# Autodesk Inventor assembly: basic c-channel design
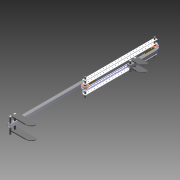
[picture p0: Inventor's stored thumbnail of the model, 180x180]
Saved by Autodesk Inventor 2011 (Build 150239000, 239)
## iProperties
Created: 2013-01-27
Part Number: basic c-channel design
Document SubType Name: Assembly
Designer: Danny
Author: Danny
## Documents named in this file (18)
- C:\Users\Danny\Documents\GitHub\2013CAD\2013 robot\hybrid climber designs\spiderfork\basic c-channel design.iam
- C:\Users\Danny\Documents\GitHub\2013CAD\2013 robot\hybrid climber designs\spiderfork\c-channel (24 in with .5 in holes).ipt
- C:\Users\Danny\Documents\GitHub\2013CAD\2013 robot\hybrid climber designs\spiderfork\axle.ipt
- C:\Users\Danny\Documents\GitHub\2013CAD\2013 robot\hybrid climber designs\spiderfork\tiny dual sprocket.ipt
- C:\Users\Danny\Documents\GitHub\2013CAD\2013 robot\hybrid climber designs\spiderfork\axle spacer.ipt
- C:\Users\Danny\Documents\GitHub\2013CAD\2013 robot\hybrid climber designs\spiderfork\false chain.ipt
- C:\Users\Danny\Documents\GitHub\2013CAD\2013 robot\hybrid climber designs\spiderfork\26 in 1-16 tubing.ipt
- C:\Users\Danny\Documents\GitHub\2013CAD\2013 robot\hybrid climber designs\spiderfork\imaginary stopper.ipt
- C:\Users\Danny\Documents\GitHub\2013CAD\2013 robot\hybrid climber designs\spiderfork\long hex bolt.ipt
- C:\Users\Danny\Documents\GitHub\2013CAD\2013 robot\hybrid climber designs\spiderfork\nylock nut.ipt
- C:\Users\Danny\Documents\GitHub\2013CAD\2013 robot\hybrid climber designs\spiderfork\lexan bolt spacer.ipt
- C:\Users\Danny\Documents\GitHub\2013CAD\2013 robot\hybrid climber designs\spiderfork\lexan stop bolt spacer.ipt
- C:\Users\Danny\Documents\GitHub\2013CAD\2013 robot\hybrid climber designs\spiderfork\4 in 1-16 tubing.ipt
- C:\Users\Danny\Documents\GitHub\2013CAD\2013 robot\hybrid climber designs\spiderfork\lexan stuff (bottom).ipt
- C:\Users\Danny\Documents\GitHub\2013CAD\2013 robot\hybrid climber designs\spiderfork\very long hex bolt.ipt
- C:\Users\Danny\Documents\GitHub\2013CAD\2013 robot\hybrid climber designs\spiderfork\lexan stuff.ipt
- C:\Users\Danny\Documents\GitHub\2013CAD\2013 robot\hybrid climber designs\spiderfork\lexan top bolt spacer.ipt
- C:\Users\Danny\Documents\GitHub\2013CAD\2013 robot\hybrid climber designs\spiderfork\lexan top bolt stop spacer.ipt
## Components (36 placed, 16 different names)
1. c-channel (24 in with .5 in holes):1 — Mate:2, Mate:3, Mate:12, Mate:17
2. c-channel (24 in with .5 in holes):2 — Mate:1, Mate:4, Mate:9
3. axle:1 — Mate:1, Mate:2, Mate:5, Mate:7, Mate:8
4. axle:2 — Mate:3, Mate:4, Mate:6, Mate:13, Mate:14
5. tiny dual sprocket:1 — Mate:5, Mate:10, Mate:11, Mate:19, Mate:21, Flush:1, Flush:2
6. tiny dual sprocket:2 — Mate:6, Mate:15, Mate:16, Mate:18, Mate:20
7. axle spacer:1 — Mate:14, Mate:16
8. axle spacer:2 — Mate:13, Mate:15, Mate:17
9. axle spacer:3 — Mate:8, Mate:11, Mate:12
10. axle spacer:4 — Mate:7, Mate:9, Mate:10
11. false chain:1 — Mate:18, Mate:19, Flush:1, Mate:25, Mate:50, Mate:51, Mate:53, Mate:54, Mate:55
12. false chain:2 — Mate:20, Mate:21, Flush:2
13. 4 in 1-16 tubing:1 — Mate:50, Flush:7, Flush:9, Mate:86
14. imaginary stopper:1 — Mate:25, Mate:51, Flush:7, Flush:9
15. lexan stuff (bottom):2 — Mate:33, Mate:43, Mate:84, Mate:85, Mate:87, Flush:14
16. lexan stuff (bottom):1 — Mate:80, Mate:81, Mate:82, Mate:88, Flush:14
17. Chassis_HexBolt_375x16x7_AndyMark_am-1055:1 — Mate:32, Mate:38, Mate:41, Mate:82, Mate:86, Mate:87, Mate:88
18. Chassis_HexBolt_375x16x7_AndyMark_am-1055:2 — Mate:36, Mate:44, Mate:45, Mate:47
19. nylock nut:1 — Mate:32, Mate:33, Mate:84
20. nylock nut:2 — Mate:36, Mate:48
21. lexan bolt spacer:1 — Mate:38, Mate:80, Mate:81
22. lexan bolt spacer:2 — Mate:41, Mate:43, Mate:85
23. lexan stop bolt spacer:1 — Mate:47, Mate:48
24. lexan stop bolt spacer:2 — Mate:44, Mate:45
25. 26 in 1-16 tubing:1 — Mate:53, Flush:8, Flush:10, Flush:11, Flush:12, Mate:59, Mate:63, Mate:65, Mate:69, Mate:70, Mate:73, Mate:75
26. imaginary stopper:2 — Mate:54, Mate:55, Flush:8, Flush:10
27. Chassis_HexBolt_375x16x7_AndyMark_am-1055:3 — Mate:58, Mate:59, Mate:60, Mate:61, Mate:64, Mate:67, Mate:79
28. Chassis_HexBolt_375x16x7_AndyMark_am-1055:4 — Mate:69, Mate:70, Mate:71, Mate:72, Mate:74, Mate:76
29. nylock nut:3 — Mate:67
30. nylock nut:4 — Mate:76, Mate:77
31. lexan stuff:1 — Flush:12, Mate:78, Mate:79, Flush:13
32. lexan stuff:2 — Flush:11, Mate:58, Mate:61, Mate:62, Flush:13
33. lexan top bolt spacer:1 — Mate:64, Mate:65, Mate:78
34. lexan top bolt spacer:2 — Mate:60, Mate:62, Mate:63
35. lexan top bolt stop spacer:1 — Mate:74, Mate:75, Mate:77
36. lexan top bolt stop spacer:2 — Mate:71, Mate:72, Mate:73
## Relationships (82: Mate 70, Flush 12)
- Mate:1: c-channel (24 in with .5 in holes):2 ↔ axle:1
- Mate:2: c-channel (24 in with .5 in holes):1 ↔ axle:1
- Mate:3: c-channel (24 in with .5 in holes):1 ↔ axle:2
- Mate:4: c-channel (24 in with .5 in holes):2 ↔ axle:2
- Mate:5: axle:1 ↔ tiny dual sprocket:1
- Mate:6: axle:2 ↔ tiny dual sprocket:2
- Mate:7: axle:1 ↔ axle spacer:4
- Mate:8: axle:1 ↔ axle spacer:3
- Mate:9: c-channel (24 in with .5 in holes):2 ↔ axle spacer:4
- Mate:10: tiny dual sprocket:1 ↔ axle spacer:4
- Mate:11: tiny dual sprocket:1 ↔ axle spacer:3
- Mate:12: c-channel (24 in with .5 in holes):1 ↔ axle spacer:3
- Mate:13: axle:2 ↔ axle spacer:2
- Mate:14: axle:2 ↔ axle spacer:1
- Mate:15: tiny dual sprocket:2 ↔ axle spacer:2
- Mate:16: tiny dual sprocket:2 ↔ axle spacer:1
- Mate:17: c-channel (24 in with .5 in holes):1 ↔ axle spacer:2
- Mate:18: tiny dual sprocket:2 ↔ false chain:1
- Mate:19: tiny dual sprocket:1 ↔ false chain:1
- Mate:20: tiny dual sprocket:2 ↔ false chain:2
- Mate:21: tiny dual sprocket:1 ↔ false chain:2
- Flush:1: tiny dual sprocket:1 ↔ false chain:1
- Flush:2: tiny dual sprocket:1 ↔ false chain:2
- Mate:25: false chain:1 ↔ imaginary stopper:1
- [Flush]: 4 in 1-16 tubing:1 ↔ lexan stuff (bottom):2
- [Flush]: 4 in 1-16 tubing:1 ↔ lexan stuff (bottom):1
- Mate:32: Chassis_HexBolt_375x16x7_AndyMark_am-1055:1 ↔ nylock nut:1
- Mate:33: lexan stuff (bottom):2 ↔ nylock nut:1
- [Mate]: 4 in 1-16 tubing:1 ↔ Chassis_HexBolt_375x16x7_AndyMark_am-1055:2
- Mate:36: Chassis_HexBolt_375x16x7_AndyMark_am-1055:2 ↔ nylock nut:2
- Mate:38: Chassis_HexBolt_375x16x7_AndyMark_am-1055:1 ↔ lexan bolt spacer:1
- [Mate]: 4 in 1-16 tubing:1 ↔ lexan bolt spacer:1
- Mate:41: Chassis_HexBolt_375x16x7_AndyMark_am-1055:1 ↔ lexan bolt spacer:2
- [Mate]: 4 in 1-16 tubing:1 ↔ lexan bolt spacer:2
- Mate:43: lexan stuff (bottom):2 ↔ lexan bolt spacer:2
- Mate:44: Chassis_HexBolt_375x16x7_AndyMark_am-1055:2 ↔ lexan stop bolt spacer:2
- Mate:45: Chassis_HexBolt_375x16x7_AndyMark_am-1055:2 ↔ lexan stop bolt spacer:2
- [Mate]: 4 in 1-16 tubing:1 ↔ lexan stop bolt spacer:2
- Mate:47: Chassis_HexBolt_375x16x7_AndyMark_am-1055:2 ↔ lexan stop bolt spacer:1
- Mate:48: nylock nut:2 ↔ lexan stop bolt spacer:1
- [Mate]: 4 in 1-16 tubing:1 ↔ lexan stop bolt spacer:1
- Mate:50: false chain:1 ↔ 4 in 1-16 tubing:1
- Mate:51: false chain:1 ↔ imaginary stopper:1
- Flush:7: 4 in 1-16 tubing:1 ↔ imaginary stopper:1
- Mate:53: false chain:1 ↔ 26 in 1-16 tubing:1
- Mate:54: false chain:1 ↔ imaginary stopper:2
- Mate:55: false chain:1 ↔ imaginary stopper:2
- Flush:8: 26 in 1-16 tubing:1 ↔ imaginary stopper:2
- Flush:9: 4 in 1-16 tubing:1 ↔ imaginary stopper:1
- Flush:10: 26 in 1-16 tubing:1 ↔ imaginary stopper:2
- Flush:11: 26 in 1-16 tubing:1 ↔ lexan stuff:2
- Flush:12: 26 in 1-16 tubing:1 ↔ lexan stuff:1
- Mate:58: Chassis_HexBolt_375x16x7_AndyMark_am-1055:3 ↔ lexan stuff:2
- Mate:59: 26 in 1-16 tubing:1 ↔ Chassis_HexBolt_375x16x7_AndyMark_am-1055:3
- Mate:60: Chassis_HexBolt_375x16x7_AndyMark_am-1055:3 ↔ lexan top bolt spacer:2
- Mate:61: Chassis_HexBolt_375x16x7_AndyMark_am-1055:3 ↔ lexan stuff:2
- Mate:62: lexan stuff:2 ↔ lexan top bolt spacer:2
- Mate:63: 26 in 1-16 tubing:1 ↔ lexan top bolt spacer:2
- Mate:64: Chassis_HexBolt_375x16x7_AndyMark_am-1055:3 ↔ lexan top bolt spacer:1
- Mate:65: 26 in 1-16 tubing:1 ↔ lexan top bolt spacer:1
- Mate:67: Chassis_HexBolt_375x16x7_AndyMark_am-1055:3 ↔ nylock nut:3
- Mate:69: 26 in 1-16 tubing:1 ↔ Chassis_HexBolt_375x16x7_AndyMark_am-1055:4
- Mate:70: 26 in 1-16 tubing:1 ↔ Chassis_HexBolt_375x16x7_AndyMark_am-1055:4
- Mate:71: Chassis_HexBolt_375x16x7_AndyMark_am-1055:4 ↔ lexan top bolt stop spacer:2
- Mate:72: Chassis_HexBolt_375x16x7_AndyMark_am-1055:4 ↔ lexan top bolt stop spacer:2
- Mate:73: 26 in 1-16 tubing:1 ↔ lexan top bolt stop spacer:2
- Mate:74: Chassis_HexBolt_375x16x7_AndyMark_am-1055:4 ↔ lexan top bolt stop spacer:1
- Mate:75: 26 in 1-16 tubing:1 ↔ lexan top bolt stop spacer:1
- Mate:76: Chassis_HexBolt_375x16x7_AndyMark_am-1055:4 ↔ nylock nut:4
- Mate:77: nylock nut:4 ↔ lexan top bolt stop spacer:1
- Mate:78: lexan stuff:1 ↔ lexan top bolt spacer:1
- Mate:79: Chassis_HexBolt_375x16x7_AndyMark_am-1055:3 ↔ lexan stuff:1
- Flush:13: lexan stuff:1 ↔ lexan stuff:2
- Mate:80: lexan stuff (bottom):1 ↔ lexan bolt spacer:1
- Mate:81: lexan stuff (bottom):1 ↔ lexan bolt spacer:1
- Mate:82: lexan stuff (bottom):1 ↔ Chassis_HexBolt_375x16x7_AndyMark_am-1055:1
- Mate:84: lexan stuff (bottom):2 ↔ nylock nut:1
- Mate:85: lexan stuff (bottom):2 ↔ lexan bolt spacer:2
- Mate:86: 4 in 1-16 tubing:1 ↔ Chassis_HexBolt_375x16x7_AndyMark_am-1055:1
- Mate:87: lexan stuff (bottom):2 ↔ Chassis_HexBolt_375x16x7_AndyMark_am-1055:1
- Mate:88: lexan stuff (bottom):1 ↔ Chassis_HexBolt_375x16x7_AndyMark_am-1055:1
- Flush:14: lexan stuff (bottom):2 ↔ lexan stuff (bottom):1
